# Autodesk Inventor assembly: teljes3
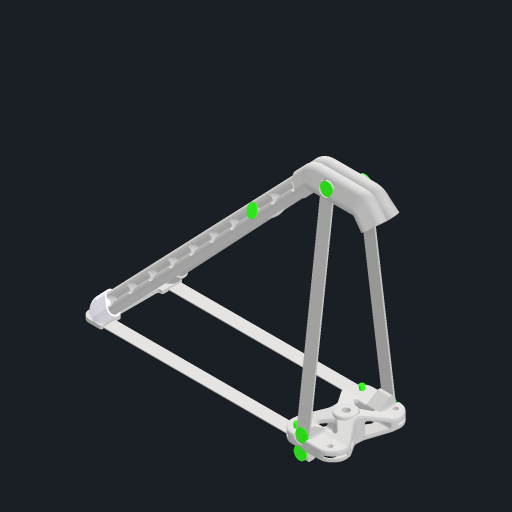
[picture p0: Inventor's stored thumbnail of the model, 512x512]
Saved by Autodesk Inventor 2023 (Build 270158000, 158)
## iProperties
Created: 2022-11-11
Part Number: teljes3
Document SubType Name: Assembly
Designer: gd1
Author: gd1
## Documents named in this file (10)
- C:\Users\gd1\3D Objects\3D nagyteherbírású híd\Híd\H-d\teljes8.iam
- C:\Users\gd1\3D Objects\3D nagyteherbírású híd\Híd\H-d\45 fok középre_talp másolata.ipt
- C:\Users\gd1\3D Objects\3D nagyteherbírású híd\Híd\H-d\palca 325mm.ipt
- C:\Users\gd1\3D Objects\3D nagyteherbírású híd\Híd\H-d\tipli.ipt
- C:\Users\gd1\3D Objects\3D nagyteherbírású híd\Híd\H-d\kozepso_csomopont3.1 másolata.ipt
- C:\Users\gd1\3D Objects\3D nagyteherbírású híd\Híd\H-d\osszekotoelem.iam
- C:\Users\gd1\3D Objects\3D nagyteherbírású híd\Híd\H-d\kozepso szalag2.ipt
- C:\Users\gd1\3D Objects\3D nagyteherbírású híd\Híd\H-d\45 fok kozepcsati.ipt.iam
- C:\Users\gd1\3D Objects\3D nagyteherbírású híd\Híd\H-d\közepső szalag 1.ipt
- 45 fok kozepcsati.ipt
## Components (22 placed, 8 different names)
1. 45 fok középre_talp másolata:1 — Rotational:1, Rotational:2, Rotational:14, Rotational:15
2. palca 325mm:1 — Rotational:1, Insert:1
3. palca 325mm:2 — Rotational:2, Rotational:17
4. tipli:9
5. tipli:10
6. kozepso_csomopont3.1 másolata:1 — Rotational:16, Rotational:18, Rotational:19
7. osszekotoelem:1 [sub-assembly] — Insert:1, Rotational:12, Rotational:13
8. tipli:11 — Rotational:12
9. tipli:12 — Rotational:13
10. kozepso szalag2:2 — Rotational:15, Rotational:23
11. kozepso szalag2:3 — Rotational:14, Rotational:16, Rotational:22
12. 45 fok kozepcsati.ipt:1 [sub-assembly] — Rotational:17, Rotational:27, Rotational:28
13. közepső szalag 1:2 — Rotational:18, Rigid:1, Rotational:20, Rotational:21, Rotational:27
14. közepső szalag 1:3 — Rotational:19, Rotational:24, Rotational:25, Rotational:26, Rotational:28
15. tipli:13 — Rigid:1
16. tipli:14 — Rotational:20
17. tipli:15 — Rotational:21
18. tipli:16 — Rotational:22
19. tipli:17 — Rotational:23
20. tipli:18 — Rotational:24
21. tipli:19 — Rotational:25
22. tipli:20 — Rotational:26
## Relationships (21: RevoluteJoint 19, Insert 1, WeldJoint 1)
- Rotational:1 [RevoluteJoint]: 45 fok középre_talp másolata:1 ↔ palca 325mm:1
- Rotational:2 [RevoluteJoint]: 45 fok középre_talp másolata:1 ↔ palca 325mm:2
- Insert:1: palca 325mm:1 ↔ osszekotoelem:1
- Rotational:12 [RevoluteJoint]: osszekotoelem:1 ↔ tipli:11
- Rotational:13 [RevoluteJoint]: osszekotoelem:1 ↔ tipli:12
- Rotational:14 [RevoluteJoint]: 45 fok középre_talp másolata:1 ↔ kozepso szalag2:3
- Rotational:15 [RevoluteJoint]: 45 fok középre_talp másolata:1 ↔ kozepso szalag2:2
- Rotational:16 [RevoluteJoint]: kozepso_csomopont3.1 másolata:1 ↔ kozepso szalag2:3
- Rotational:17 [RevoluteJoint]: palca 325mm:2 ↔ 45 fok kozepcsati.ipt:1
- Rotational:18 [RevoluteJoint]: kozepso_csomopont3.1 másolata:1 ↔ közepső szalag 1:2
- Rotational:19 [RevoluteJoint]: kozepso_csomopont3.1 másolata:1 ↔ közepső szalag 1:3
- Rigid:1 [WeldJoint]: közepső szalag 1:2 ↔ tipli:13
- Rotational:20 [RevoluteJoint]: közepső szalag 1:2 ↔ tipli:14
- Rotational:21 [RevoluteJoint]: közepső szalag 1:2 ↔ tipli:15
- Rotational:22 [RevoluteJoint]: kozepso szalag2:3 ↔ tipli:16
- Rotational:23 [RevoluteJoint]: kozepso szalag2:2 ↔ tipli:17
- Rotational:24 [RevoluteJoint]: közepső szalag 1:3 ↔ tipli:18
- Rotational:25 [RevoluteJoint]: közepső szalag 1:3 ↔ tipli:19
- Rotational:26 [RevoluteJoint]: közepső szalag 1:3 ↔ tipli:20
- Rotational:27 [RevoluteJoint]: 45 fok kozepcsati.ipt:1 ↔ közepső szalag 1:2
- Rotational:28 [RevoluteJoint]: 45 fok kozepcsati.ipt:1 ↔ közepső szalag 1:3
